# Autodesk Inventor assembly: Krasser Roboter weniger Gewindestangen
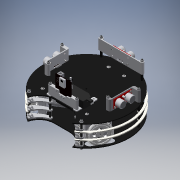
[picture p0: Inventor's stored thumbnail of the model, 180x180]
Saved by Autodesk Inventor 2018 (Build 220112000, 112)
## iProperties
Created: 2019-03-04
Part Number: Krasser Roboter weniger Gewindestangen
Material: Generisch
Document SubType Name: Assembly
Designer: RedBots
Mass: 1105.68 g
Surface Area: 3152.09 cm^2
Volume: 618.707 cm^3
Density: 1.78708 g/cm^3
Author: RedBots
## Documents named in this file (37)
- C:\Users\RedBots\Desktop\FinalRobot\Krasser Roboter weniger Gewindestangen.iam
- C:\Users\RedBots\Desktop\FinalRobot\Bodenplatine.ipt
- C:\Users\RedBots\Desktop\FinalRobot\alu_ring_pesus.ipt
- C:\Users\RedBots\Desktop\FinalRobot\Fake Rad.ipt
- C:\Users\RedBots\Desktop\FinalRobot\Hauptplatine.ipt
- C:\Users\RedBots\Desktop\FinalRobot\Akku.ipt
- C:\Users\RedBots\Desktop\FinalRobot\Akkuhalterung.ipt
- C:\Users\RedBots\Desktop\FinalRobot\Schraube M3x8 SK.ipt
- C:\Users\RedBots\Desktop\FinalRobot\Motor\Motormaxon_PN_B7453F27107C.iam
- C:\Users\RedBots\Desktop\FinalRobot\LED 3mm.ipt
- C:\Users\RedBots\Desktop\FinalRobot\Halterung Lichtschranke rechts.ipt
- C:\Users\RedBots\Desktop\FinalRobot\Ball.ipt
- C:\Users\RedBots\Desktop\FinalRobot\Halterung Lichtschranke links.ipt
- C:\Users\RedBots\Desktop\FinalRobot\SRF08.ipt
- C:\Users\RedBots\Desktop\FinalRobot\Pinhead 5.ipt
- C:\Users\RedBots\Desktop\FinalRobot\Schraube M3x8 LK.ipt
- C:\Users\RedBots\Desktop\FinalRobot\US Halterung rechts.ipt
- C:\Users\RedBots\Desktop\FinalRobot\US Halterung links.ipt
- C:\Users\RedBots\Desktop\FinalRobot\Pixy 2.iam
- C:\Users\RedBots\Desktop\FinalRobot\Pixy 2 Halterung.ipt
- C:\Users\RedBots\Desktop\FinalRobot\Abstandshalter US Sensor.ipt
- C:\Users\RedBots\Desktop\FinalRobot\Scheibe M3 Polyamid.ipt
- C:\Users\RedBots\Desktop\FinalRobot\Sicherungsmutter M3.ipt
- C:\Users\RedBots\Desktop\FinalRobot\Schraube M3x16 LK.ipt
- C:\Users\RedBots\Desktop\FinalRobot\US Halterung hinten leicht.ipt
- C:\Users\RedBots\Desktop\FinalRobot\Gewindestange M3x103mm.ipt
- C:\Users\RedBots\Desktop\FinalRobot\Abstandshalter 15mm leicht.ipt
- C:\Users\RedBots\Desktop\FinalRobot\Abstandshalter 12mm leicht.ipt
- C:\Users\RedBots\Desktop\FinalRobot\Abstandshalter 3mm.ipt
- C:\Users\RedBots\Desktop\FinalRobot\Gewindestange M3x91mm.ipt
- C:\Users\RedBots\Desktop\FinalRobot\Gewindestange M3x63mm.ipt
- C:\Users\RedBots\Desktop\FinalRobot\Abstandshalter 14mm leicht.ipt
- C:\Users\RedBots\Desktop\FinalRobot\Gewindestange M3x85mm.ipt
- C:\Users\RedBots\Desktop\FinalRobot\Schraube M3x12 LK.ipt
- C:\Users\RedBots\Desktop\FinalRobot\Motorhalterung leicht H.ipt
- C:\Users\RedBots\Desktop\FinalRobot\Motorhalterung leicht VL.ipt
- C:\Users\RedBots\Desktop\FinalRobot\Motorhalterung leicht VR.ipt
## Components (151 placed, 37 different names)
1. Ball:1 — Passend:142, Passend:143
2. Abstandshalter 3mm:1 — Passend:322, Passend:328
3. Abstandshalter 3mm:2 — Passend:330, Passend:331, Passend:332
4. Abstandshalter 3mm:3 — Passend:337, Passend:339
5. Abstandshalter 3mm:4 — Passend:338, Passend:340, Passend:341
6. Gewindestange M3x91mm:1 — Passend:323, Passend:324, Fluchtend:31, Passend:325, Passend:326, Passend:329, Passend:330, Passend:333
7. Sicherungsmutter M3:15 — Passend:326, Passend:327
8. Sicherungsmutter M3:16 — Passend:333, Passend:336
9. Sicherungsmutter M3:17 — Passend:334, Passend:335
10. Sicherungsmutter M3:18 — Passend:342, Passend:344
11. Sicherungsmutter M3:19 — Passend:343, Passend:345
12. Abstandshalter 15mm leicht:13 — Passend:347, Passend:349
13. Abstandshalter 15mm leicht:14 — Passend:346, Passend:348, Passend:350
14. Sicherungsmutter M3:20 — Passend:351, Passend:353
15. Sicherungsmutter M3:21 — Passend:352, Passend:354
16. Schraube M3x16 LK:4 — Passend:355, Passend:356, Passend:357, Passend:358
17. Schraube M3x16 LK:5 — Passend:359, Passend:360, Passend:361, Passend:362
18. Schraube M3x16 LK:6 — Passend:363, Passend:364, Passend:365
19. Schraube M3x16 LK:7 — Passend:366, Passend:367, Passend:368
20. Sicherungsmutter M3:22 — Passend:370, Passend:372
21. Sicherungsmutter M3:23 — Passend:369, Passend:371
22. Abstandshalter 12mm leicht:7 — Passend:373, Passend:375
23. Abstandshalter 12mm leicht:8 — Passend:374, Passend:376, Passend:377
24. Abstandshalter 14mm leicht:1 — Passend:380, Passend:382
25. Abstandshalter 14mm leicht:2 — Passend:379, Passend:385, Passend:387
26. Abstandshalter 14mm leicht:3 — Passend:378, Passend:384, Passend:386
27. Abstandshalter 14mm leicht:4 — Passend:381, Passend:383
28. Sicherungsmutter M3:24 — Passend:389, Passend:391
29. Sicherungsmutter M3:25 — Passend:390, Passend:392
30. Schraube M3x16 LK:8 — Passend:399, Passend:400
31. Schraube M3x16 LK:9 — Passend:393, Passend:394, Passend:397
32. Scheibe M3 Polyamid:27 — Passend:395, Passend:396, Passend:397
33. Sicherungsmutter M3:26 — Passend:405, Passend:408
34. Sicherungsmutter M3:27 — Passend:404, Passend:407
35. Sicherungsmutter M3:28 — Passend:406, Passend:409
36. Bodenplatine:1 — Passend:17, Fluchtend:2, Passend:18, Passend:21, Passend:24, Passend:25, Passend:26, Passend:27, Passend:28, Passend:29, Passend:30, Passend:31, Passend:32, Fluchtend:7, Fluchtend:8, Fluchtend:9, Fluchtend:10, Fluchtend:11, Fluchtend:12, Fluchtend:13, Fluchtend:14, Passend:100, Passend:102, Passend:105, Passend:106, Passend:143, Passend:157, Passend:158, Passend:262, Passend:263, Passend:264, Passend:265, Passend:266, Passend:267, Passend:268, Passend:269, Passend:270, Passend:271, Passend:272, Passend:273, Passend:274, Passend:275, Passend:324, Fluchtend:31, Passend:367, Passend:398
37. Hauptplatine:1 — Passend:48, Passend:49, Passend:50, Passend:53, Passend:54, Passend:61, Passend:63, Passend:238, Passend:241, Passend:243, Passend:245, Passend:247, Passend:331, Passend:339, Passend:340, Passend:348, Passend:349, Passend:355, Passend:361, Passend:375, Passend:376, Passend:394, Passend:395, Passend:396
38. Gewindestange M3x85mm:2 — Passend:28, Fluchtend:8, Passend:62, Passend:128, Passend:137, Passend:140, Passend:209, Passend:250, Passend:293, Passend:374, Passend:380, Passend:381, Passend:390
39. Gewindestange M3x85mm:1 — Passend:26, Fluchtend:9, Passend:60, Passend:130, Passend:134, Passend:138, Passend:208, Passend:261, Passend:276, Passend:373, Passend:378, Passend:379, Passend:389
40. Gewindestange M3x91mm:3 — Passend:13, Passend:17, Fluchtend:2, Passend:179, Passend:258, Passend:292, Passend:338, Passend:343
41. Gewindestange M3x63mm:1 — Passend:25, Fluchtend:10, Passend:33, Passend:36, Passend:49, Passend:86, Passend:87, Passend:112, Passend:131, Passend:135, Passend:139, Passend:234, Passend:260, Passend:298, Passend:370
42. Gewindestange M3x63mm:2 — Passend:29, Fluchtend:7, Passend:34, Passend:37, Passend:50, Passend:92, Passend:93, Passend:113, Passend:129, Passend:136, Passend:141, Passend:227, Passend:248, Passend:300, Passend:369
43. Gewindestange M3x91mm:2 — Passend:30, Fluchtend:14, Passend:94, Passend:95, Passend:114, Passend:204, Passend:252, Passend:280, Passend:322, Passend:334
44. Gewindestange M3x103mm:1 — Passend:32, Fluchtend:12, Passend:90, Passend:91, Passend:116, Passend:256, Passend:288, Passend:317, Passend:347, Passend:352
45. Gewindestange M3x103mm:2 — Passend:31, Fluchtend:13, Passend:96, Passend:97, Passend:117, Passend:253, Passend:285, Passend:316, Passend:346, Passend:351
46. Gewindestange M3x91mm:4 — Passend:27, Fluchtend:11, Passend:88, Passend:89, Passend:115, Passend:180, Passend:257, Passend:289, Passend:337, Passend:342
47. Ring unten — Passend:33, Passend:34, Passend:101, Passend:103, Passend:104, Passend:107, Passend:110, Passend:156, Passend:159
48. Ring oben — Passend:36, Passend:37, Passend:111, Passend:118, Passend:119, Passend:120, Passend:121, Passend:132, Passend:133
49. Fake Rad:1 — Tangential:2, Passend:75, Fluchtend:23
50. Fake Rad:2 — Tangential:1, Passend:70, Fluchtend:22
51. Fake Rad:3 — Passend:76, Fluchtend:24
52. Akku:1 — Passend:59, Passend:64, Fluchtend:18
53. Akkuhalterung:1 — Passend:54, Passend:62, Passend:63
54. Akkuhalterung:2 — Passend:53, Passend:59, Passend:60, Passend:61, Passend:64, Fluchtend:18, Passend:388
55. Motormaxon_PN_B7453F27107C:3 [sub-assembly] — Passend:68, Passend:69, Passend:70, Fluchtend:22, Passend:85
56. Motormaxon_PN_B7453F27107C:1 [sub-assembly] — Passend:71, Passend:72, Passend:75, Fluchtend:23, Passend:84
57. Motormaxon_PN_B7453F27107C:2 [sub-assembly] — Passend:73, Passend:74, Passend:76, Fluchtend:24, Passend:80, Passend:81, Passend:82, Passend:83
58. Abstandshalter 12mm leicht:1 — Passend:86, Passend:98
59. Abstandshalter 12mm leicht:2 — Passend:87, Passend:99
60. Abstandshalter 12mm leicht:3 — Passend:93, Passend:109
61. Abstandshalter 12mm leicht:4 — Passend:92, Passend:108, Passend:110
62. Abstandshalter 12mm leicht:5 — Passend:112, Passend:122
63. Abstandshalter 12mm leicht:6 — Passend:113, Passend:123
64. Abstandshalter 15mm leicht:1 — Passend:97, Passend:104
65. Abstandshalter 15mm leicht:2 — Passend:95, Passend:107, Passend:111
66. Abstandshalter 15mm leicht:3 — Passend:96, Passend:105
67. Abstandshalter 15mm leicht:4 — Passend:94, Passend:106
68. Abstandshalter 15mm leicht:5 — Passend:88, Passend:101
69. Abstandshalter 15mm leicht:6 — Passend:89, Passend:100
70. Abstandshalter 15mm leicht:7 — Passend:90, Passend:102
71. Abstandshalter 15mm leicht:8 — Passend:91, Passend:103
72. Abstandshalter 15mm leicht:9 — Passend:115, Passend:121
73. Abstandshalter 15mm leicht:10 — Passend:114, Passend:119
74. Abstandshalter 15mm leicht:11 — Passend:116, Passend:120
75. Abstandshalter 15mm leicht:12 — Passend:117, Passend:118
76. Halterung Lichtschranke links:1 — Passend:130, Passend:131, Passend:132, Passend:144, Passend:145, Passend:122, Passend:384
77. Halterung Lichtschranke links:2 — Passend:134, Passend:135, Passend:146, Passend:154, Passend:156, Passend:99, Passend:385, Passend:386
78. Halterung Lichtschranke rechts:2 — Passend:136, Passend:137, Passend:149, Passend:152, Passend:159, Passend:109, Passend:383
79. Halterung Lichtschranke links:3 — Passend:138, Passend:139, Passend:147, Passend:155, Passend:157, Passend:98, Passend:387
80. Halterung Lichtschranke rechts:3 — Passend:140, Passend:141, Passend:150, Passend:153, Passend:158, Passend:108
81. Halterung Lichtschranke rechts:1 — Passend:128, Passend:129, Passend:133, Passend:148, Passend:151, Passend:123, Passend:377, Passend:382
82. LED 3mm:1 — Passend:144, Passend:145
83. LED 3mm:2 — Passend:150, Passend:153
84. LED 3mm:3 — Passend:149, Passend:152
85. LED 3mm:4 — Passend:147, Passend:155
86. LED 3mm:5 — Passend:146, Passend:154
87. LED 3mm:6 — Passend:148, Passend:151
88. Schraube M3x12 LK:3 — Passend:402, Passend:406
89. Schraube M3x12 LK:2 — Passend:403, Passend:405
90. Schraube M3x12 LK:1 — Passend:401, Passend:404
91. Pixy 2 Halterung:1 — Passend:208, Passend:209, Passend:212, Passend:213, Passend:214, Passend:215, Passend:402, Passend:403, Passend:388, Passend:391, Passend:392, Passend:401, Passend:407, Passend:408, Passend:409
92. Pixy 2:2 [sub-assembly] — Passend:212, Passend:213, Passend:214, Passend:215
93. Scheibe M3 Polyamid:3 — Passend:227, Passend:243, Passend:371
94. Scheibe M3 Polyamid:4 — Passend:234, Passend:238, Passend:372
95. Scheibe M3 Polyamid:7 — Passend:247, Passend:360, Passend:362
96. Scheibe M3 Polyamid:8 — Passend:245, Passend:357, Passend:358
97. Scheibe M3 Polyamid:10 — Passend:241, Passend:315
98. Scheibe M3 Polyamid:13 — Passend:265, Passend:325, Passend:327
99. Scheibe M3 Polyamid:14 — Passend:256, Passend:270, Passend:291
100. Scheibe M3 Polyamid:15 — Passend:248, Passend:262, Passend:303
101. Scheibe M3 Polyamid:16 — Passend:263, Passend:313
102. Scheibe M3 Polyamid:17 — Passend:260, Passend:275, Passend:301
103. Scheibe M3 Polyamid:18 — Passend:261, Passend:273, Passend:277
104. Scheibe M3 Polyamid:19 — Passend:258, Passend:272, Passend:295
105. Scheibe M3 Polyamid:20 — Passend:268, Passend:364, Passend:365
106. Scheibe M3 Polyamid:21 — Passend:269, Passend:366, Passend:368
107. Scheibe M3 Polyamid:22 — Passend:253, Passend:267, Passend:287
108. Scheibe M3 Polyamid:23 — Passend:274, Passend:398, Passend:399, Passend:400
109. Scheibe M3 Polyamid:24 — Passend:257, Passend:271, Passend:290
110. Scheibe M3 Polyamid:25 — Passend:252, Passend:266, Passend:282
111. Scheibe M3 Polyamid:26 — Passend:250, Passend:264, Passend:294
112. Sicherungsmutter M3:1 — Passend:288, Passend:291
113. Sicherungsmutter M3:2 — Passend:289, Passend:290
114. Sicherungsmutter M3:4 — Passend:285, Passend:287
115. Sicherungsmutter M3:6 — Passend:276, Passend:277
116. Sicherungsmutter M3:7 — Passend:280, Passend:282
117. Sicherungsmutter M3:10 — Passend:293, Passend:294
118. Sicherungsmutter M3:11 — Passend:292, Passend:295
119. Sicherungsmutter M3:12 — Passend:298, Passend:301
120. Sicherungsmutter M3:14 — Passend:300, Passend:303
121. Schraube M3x8 SK:1 — Fluchtend:19, Passend:67
122. Schraube M3x8 SK:2 — Fluchtend:20, Passend:66
123. Schraube M3x8 SK:3 — Fluchtend:21, Passend:65
124. Motorhalterung leicht VR:1 — Passend:13, Passend:18, Fluchtend:19, Fluchtend:20, Fluchtend:21, Passend:65, Passend:66, Passend:67, Passend:71, Passend:72, Passend:84, Passend:393
125. Motorhalterung leicht H:1 — Passend:24, Passend:68, Passend:69, Passend:77, Passend:78, Passend:79, Fluchtend:25, Fluchtend:26, Fluchtend:27, Passend:85, Passend:356, Passend:359, Passend:363
126. Schraube M3x8 SK:4 — Passend:77, Fluchtend:26
127. Schraube M3x8 SK:5 — Passend:78, Fluchtend:27
128. Schraube M3x8 SK:6 — Passend:79, Fluchtend:25
129. Schraube M3x16 LK:1 — Passend:313
130. Schraube M3x16 LK:3 — Passend:314, Passend:315
131. Motorhalterung leicht VL:1 — Passend:21, Passend:48, Passend:73, Passend:74, Passend:83, Fluchtend:28, Fluchtend:29, Fluchtend:30, Passend:314, Passend:323
132. Schraube M3x8 SK:7 — Passend:81, Fluchtend:28
133. Schraube M3x8 SK:8 — Passend:82, Fluchtend:30
134. Schraube M3x8 SK:9 — Passend:80, Fluchtend:29
135. Pinhead 5:1 — Passend:164, Passend:165, Passend:166
136. SRF08:3 — Passend:164, Passend:165, Passend:166, Passend:172, Passend:173, Passend:174, Passend:175, Passend:224, Passend:225
137. US Halterung hinten leicht:1 — Passend:316, Passend:317, Passend:319, Passend:320, Passend:321, Passend:350, Passend:353, Passend:354
138. Schraube M3x8 LK:1 — Passend:173, Passend:174, Passend:223, Passend:320
139. Schraube M3x8 LK:2 — Passend:172, Passend:175, Passend:222, Passend:319
140. Abstandshalter US Sensor:1 — Passend:222, Passend:224, Passend:321
141. Abstandshalter US Sensor:2 — Passend:223, Passend:225
142. SRF08:2 — Passend:182, Passend:183, Passend:184, Passend:185, Passend:186, Passend:187, Passend:188, Passend:189
143. US Halterung rechts:1 — Passend:179, Passend:180, Passend:182, Passend:190, Passend:191, Passend:341, Passend:344, Passend:345
144. Pinhead 5:2 — Passend:183, Passend:184, Passend:185
145. Schraube M3x8 LK:3 — Passend:186, Passend:188, Passend:191
146. Schraube M3x8 LK:4 — Passend:187, Passend:189, Passend:190
147. SRF08:1 — Passend:195, Passend:196, Passend:197, Passend:198, Passend:199, Passend:200, Passend:201, Passend:205
148. Pinhead 5:3 — Passend:195, Passend:196, Passend:197
149. Schraube M3x8 LK:5 — Passend:199, Passend:201, Passend:207
150. Schraube M3x8 LK:6 — Passend:198, Passend:200, Passend:206
151. US Halterung links:1 — Passend:204, Passend:205, Passend:206, Passend:207, Passend:328, Passend:329, Passend:332, Passend:335, Passend:336
## Relationships (334: Mate 309, Flush 23, Tangent 2)
- Passend:13 [Mate]: Gewindestange M3x91mm:3 ↔ Motorhalterung leicht VR:1
- Passend:17 [Mate]: Bodenplatine:1 ↔ Gewindestange M3x91mm:3
- Fluchtend:2 [Flush] (-5 mm): Bodenplatine:1 ↔ Gewindestange M3x91mm:3
- Passend:18 [Mate]: Bodenplatine:1 ↔ Motorhalterung leicht VR:1
- Passend:21 [Mate]: Bodenplatine:1 ↔ Motorhalterung leicht VL:1
- Passend:24 [Mate]: Bodenplatine:1 ↔ Motorhalterung leicht H:1
- Passend:25 [Mate]: Bodenplatine:1 ↔ Gewindestange M3x63mm:1
- Passend:26 [Mate]: Bodenplatine:1 ↔ Gewindestange M3x85mm:1
- Passend:27 [Mate]: Bodenplatine:1 ↔ Gewindestange M3x91mm:4
- Passend:28 [Mate]: Bodenplatine:1 ↔ Gewindestange M3x85mm:2
- Passend:29 [Mate]: Bodenplatine:1 ↔ Gewindestange M3x63mm:2
- Passend:30 [Mate]: Bodenplatine:1 ↔ Gewindestange M3x91mm:2
- Passend:31 [Mate]: Bodenplatine:1 ↔ Gewindestange M3x103mm:2
- Passend:32 [Mate]: Bodenplatine:1 ↔ Gewindestange M3x103mm:1
- Fluchtend:7 [Flush] (-5 mm): Bodenplatine:1 ↔ Gewindestange M3x63mm:2
- Fluchtend:8 [Flush] (5 mm): Bodenplatine:1 ↔ Gewindestange M3x85mm:2
- Fluchtend:9 [Flush] (5 mm): Bodenplatine:1 ↔ Gewindestange M3x85mm:1
- Fluchtend:10 [Flush] (5 mm): Bodenplatine:1 ↔ Gewindestange M3x63mm:1
- Fluchtend:11 [Flush] (-5 mm): Bodenplatine:1 ↔ Gewindestange M3x91mm:4
- Fluchtend:12 [Flush] (-5 mm): Bodenplatine:1 ↔ Gewindestange M3x103mm:1
- Fluchtend:13 [Flush] (-5 mm): Bodenplatine:1 ↔ Gewindestange M3x103mm:2
- Fluchtend:14 [Flush] (-5 mm): Bodenplatine:1 ↔ Gewindestange M3x91mm:2
- Passend:33 [Mate]: Gewindestange M3x63mm:1 ↔ Ring unten
- Passend:34 [Mate]: Gewindestange M3x63mm:2 ↔ Ring unten
- Passend:36 [Mate]: Gewindestange M3x63mm:1 ↔ Ring oben
- Passend:37 [Mate]: Gewindestange M3x63mm:2 ↔ Ring oben
- Passend:48 [Mate]: Hauptplatine:1 ↔ Motorhalterung leicht VL:1
- Passend:49 [Mate]: Hauptplatine:1 ↔ Gewindestange M3x63mm:1
- Passend:50 [Mate]: Hauptplatine:1 ↔ Gewindestange M3x63mm:2
- Passend:53 [Mate]: Hauptplatine:1 ↔ Akkuhalterung:2
- Passend:54 [Mate]: Hauptplatine:1 ↔ Akkuhalterung:1
- Passend:59 [Mate]: Akku:1 ↔ Akkuhalterung:2
- Passend:60 [Mate]: Gewindestange M3x85mm:1 ↔ Akkuhalterung:2
- Passend:61 [Mate]: Hauptplatine:1 ↔ Akkuhalterung:2
- Passend:62 [Mate]: Gewindestange M3x85mm:2 ↔ Akkuhalterung:1
- Passend:63 [Mate]: Hauptplatine:1 ↔ Akkuhalterung:1
- Tangential:1: Fake Rad:2
- Tangential:2: Fake Rad:1
- Passend:64 [Mate] (1.5 mm): Akku:1 ↔ Akkuhalterung:2
- Fluchtend:18 [Flush]: Akku:1 ↔ Akkuhalterung:2
- Fluchtend:19 [Flush]: Schraube M3x8 SK:1 ↔ Motorhalterung leicht VR:1
- Fluchtend:20 [Flush]: Schraube M3x8 SK:2 ↔ Motorhalterung leicht VR:1
- Fluchtend:21 [Flush]: Schraube M3x8 SK:3 ↔ Motorhalterung leicht VR:1
- Passend:65 [Mate]: Schraube M3x8 SK:3 ↔ Motorhalterung leicht VR:1
- Passend:66 [Mate]: Schraube M3x8 SK:2 ↔ Motorhalterung leicht VR:1
- Passend:67 [Mate]: Schraube M3x8 SK:1 ↔ Motorhalterung leicht VR:1
- Passend:68 [Mate]: Motormaxon_PN_B7453F27107C:3 ↔ Motorhalterung leicht H:1
- Passend:69 [Mate]: Motormaxon_PN_B7453F27107C:3 ↔ Motorhalterung leicht H:1
- Passend:70 [Mate]: Fake Rad:2 ↔ Motormaxon_PN_B7453F27107C:3
- Fluchtend:22 [Flush] (-0.5 mm): Fake Rad:2 ↔ Motormaxon_PN_B7453F27107C:3
- Passend:71 [Mate]: Motormaxon_PN_B7453F27107C:1 ↔ Motorhalterung leicht VR:1
- Passend:72 [Mate]: Motormaxon_PN_B7453F27107C:1 ↔ Motorhalterung leicht VR:1
- Passend:73 [Mate]: Motormaxon_PN_B7453F27107C:2 ↔ Motorhalterung leicht VL:1
- Passend:74 [Mate]: Motormaxon_PN_B7453F27107C:2 ↔ Motorhalterung leicht VL:1
- Passend:75 [Mate]: Fake Rad:1 ↔ Motormaxon_PN_B7453F27107C:1
- Fluchtend:23 [Flush] (0.5 mm): Fake Rad:1 ↔ Motormaxon_PN_B7453F27107C:1
- Passend:76 [Mate]: Fake Rad:3 ↔ Motormaxon_PN_B7453F27107C:2
- Fluchtend:24 [Flush] (-0.5 mm): Fake Rad:3 ↔ Motormaxon_PN_B7453F27107C:2
- Passend:77 [Mate]: Motorhalterung leicht H:1 ↔ Schraube M3x8 SK:4
- Passend:78 [Mate]: Motorhalterung leicht H:1 ↔ Schraube M3x8 SK:5
- Passend:79 [Mate]: Motorhalterung leicht H:1 ↔ Schraube M3x8 SK:6
- Fluchtend:25 [Flush]: Motorhalterung leicht H:1 ↔ Schraube M3x8 SK:6
- Fluchtend:26 [Flush]: Motorhalterung leicht H:1 ↔ Schraube M3x8 SK:4
- Fluchtend:27 [Flush]: Motorhalterung leicht H:1 ↔ Schraube M3x8 SK:5
- Passend:80 [Mate]: Motormaxon_PN_B7453F27107C:2 ↔ Schraube M3x8 SK:9
- Passend:81 [Mate]: Motormaxon_PN_B7453F27107C:2 ↔ Schraube M3x8 SK:7
- Passend:82 [Mate]: Motormaxon_PN_B7453F27107C:2 ↔ Schraube M3x8 SK:8
- Passend:83 [Mate]: Motormaxon_PN_B7453F27107C:2 ↔ Motorhalterung leicht VL:1
- Fluchtend:28 [Flush]: Motorhalterung leicht VL:1 ↔ Schraube M3x8 SK:7
- Fluchtend:29 [Flush]: Motorhalterung leicht VL:1 ↔ Schraube M3x8 SK:9
- Fluchtend:30 [Flush]: Motorhalterung leicht VL:1 ↔ Schraube M3x8 SK:8
- Passend:84 [Mate]: Motormaxon_PN_B7453F27107C:1 ↔ Motorhalterung leicht VR:1
- Passend:85 [Mate]: Motormaxon_PN_B7453F27107C:3 ↔ Motorhalterung leicht H:1
- Passend:86 [Mate]: Gewindestange M3x63mm:1 ↔ Abstandshalter 12mm leicht:1
- Passend:87 [Mate]: Gewindestange M3x63mm:1 ↔ Abstandshalter 12mm leicht:2
- Passend:88 [Mate]: Gewindestange M3x91mm:4 ↔ Abstandshalter 15mm leicht:5
- Passend:89 [Mate]: Gewindestange M3x91mm:4 ↔ Abstandshalter 15mm leicht:6
- Passend:90 [Mate]: Gewindestange M3x103mm:1 ↔ Abstandshalter 15mm leicht:7
- Passend:91 [Mate]: Gewindestange M3x103mm:1 ↔ Abstandshalter 15mm leicht:8
- Passend:92 [Mate]: Gewindestange M3x63mm:2 ↔ Abstandshalter 12mm leicht:4
- Passend:93 [Mate]: Gewindestange M3x63mm:2 ↔ Abstandshalter 12mm leicht:3
- Passend:94 [Mate]: Gewindestange M3x91mm:2 ↔ Abstandshalter 15mm leicht:4
- Passend:95 [Mate]: Gewindestange M3x91mm:2 ↔ Abstandshalter 15mm leicht:2
- Passend:96 [Mate]: Gewindestange M3x103mm:2 ↔ Abstandshalter 15mm leicht:3
- Passend:97 [Mate]: Gewindestange M3x103mm:2 ↔ Abstandshalter 15mm leicht:1
- Passend:98 [Mate]: Abstandshalter 12mm leicht:1 ↔ Halterung Lichtschranke links:3
- Passend:99 [Mate]: Abstandshalter 12mm leicht:2 ↔ Halterung Lichtschranke links:2
- Passend:100 [Mate]: Bodenplatine:1 ↔ Abstandshalter 15mm leicht:6
- Passend:101 [Mate]: Ring unten ↔ Abstandshalter 15mm leicht:5
- Passend:102 [Mate]: Bodenplatine:1 ↔ Abstandshalter 15mm leicht:7
- Passend:103 [Mate]: Ring unten ↔ Abstandshalter 15mm leicht:8
- Passend:104 [Mate]: Ring unten ↔ Abstandshalter 15mm leicht:1
- Passend:105 [Mate]: Bodenplatine:1 ↔ Abstandshalter 15mm leicht:3
- Passend:106 [Mate]: Bodenplatine:1 ↔ Abstandshalter 15mm leicht:4
- Passend:107 [Mate]: Ring unten ↔ Abstandshalter 15mm leicht:2
- Passend:108 [Mate]: Abstandshalter 12mm leicht:4 ↔ Halterung Lichtschranke rechts:3
- Passend:109 [Mate]: Abstandshalter 12mm leicht:3 ↔ Halterung Lichtschranke rechts:2
- Passend:110 [Mate]: Ring unten ↔ Abstandshalter 12mm leicht:4
- Passend:111 [Mate]: Ring oben ↔ Abstandshalter 15mm leicht:2
- Passend:112 [Mate]: Gewindestange M3x63mm:1 ↔ Abstandshalter 12mm leicht:5
- Passend:113 [Mate]: Gewindestange M3x63mm:2 ↔ Abstandshalter 12mm leicht:6
- Passend:114 [Mate]: Gewindestange M3x91mm:2 ↔ Abstandshalter 15mm leicht:10
- Passend:115 [Mate]: Gewindestange M3x91mm:4 ↔ Abstandshalter 15mm leicht:9
- Passend:116 [Mate]: Gewindestange M3x103mm:1 ↔ Abstandshalter 15mm leicht:11
- Passend:117 [Mate]: Gewindestange M3x103mm:2 ↔ Abstandshalter 15mm leicht:12
- Passend:118 [Mate]: Ring oben ↔ Abstandshalter 15mm leicht:12
- Passend:119 [Mate]: Ring oben ↔ Abstandshalter 15mm leicht:10
- Passend:120 [Mate]: Ring oben ↔ Abstandshalter 15mm leicht:11
- Passend:121 [Mate]: Ring oben ↔ Abstandshalter 15mm leicht:9
- Passend:122 [Mate]: Abstandshalter 12mm leicht:5 ↔ Halterung Lichtschranke links:1
- Passend:123 [Mate]: Abstandshalter 12mm leicht:6 ↔ Halterung Lichtschranke rechts:1
- Passend:128 [Mate]: Gewindestange M3x85mm:2 ↔ Halterung Lichtschranke rechts:1
- Passend:129 [Mate]: Gewindestange M3x63mm:2 ↔ Halterung Lichtschranke rechts:1
- Passend:130 [Mate]: Gewindestange M3x85mm:1 ↔ Halterung Lichtschranke links:1
- Passend:131 [Mate]: Gewindestange M3x63mm:1 ↔ Halterung Lichtschranke links:1
- Passend:132 [Mate]: Ring oben ↔ Halterung Lichtschranke links:1
- Passend:133 [Mate]: Ring oben ↔ Halterung Lichtschranke rechts:1
- Passend:134 [Mate]: Gewindestange M3x85mm:1 ↔ Halterung Lichtschranke links:2
- Passend:135 [Mate]: Gewindestange M3x63mm:1 ↔ Halterung Lichtschranke links:2
- Passend:136 [Mate]: Gewindestange M3x63mm:2 ↔ Halterung Lichtschranke rechts:2
- Passend:137 [Mate]: Gewindestange M3x85mm:2 ↔ Halterung Lichtschranke rechts:2
- Passend:138 [Mate]: Gewindestange M3x85mm:1 ↔ Halterung Lichtschranke links:3
- Passend:139 [Mate]: Gewindestange M3x63mm:1 ↔ Halterung Lichtschranke links:3
- Passend:140 [Mate]: Gewindestange M3x85mm:2 ↔ Halterung Lichtschranke rechts:3
- Passend:141 [Mate]: Gewindestange M3x63mm:2 ↔ Halterung Lichtschranke rechts:3
- Passend:142 [Mate] (37 mm): Ball:1
- Passend:143 [Mate] (37 mm): Ball:1 ↔ Bodenplatine:1
- Passend:144 [Mate]: Halterung Lichtschranke links:1 ↔ LED 3mm:1
- Passend:145 [Mate]: Halterung Lichtschranke links:1 ↔ LED 3mm:1
- Passend:146 [Mate]: Halterung Lichtschranke links:2 ↔ LED 3mm:5
- Passend:147 [Mate]: Halterung Lichtschranke links:3 ↔ LED 3mm:4
- Passend:148 [Mate]: Halterung Lichtschranke rechts:1 ↔ LED 3mm:6
- Passend:149 [Mate]: Halterung Lichtschranke rechts:2 ↔ LED 3mm:3
- Passend:150 [Mate]: Halterung Lichtschranke rechts:3 ↔ LED 3mm:2
- Passend:151 [Mate]: Halterung Lichtschranke rechts:1 ↔ LED 3mm:6
- Passend:152 [Mate]: Halterung Lichtschranke rechts:2 ↔ LED 3mm:3
- Passend:153 [Mate]: Halterung Lichtschranke rechts:3 ↔ LED 3mm:2
- Passend:154 [Mate]: Halterung Lichtschranke links:2 ↔ LED 3mm:5
- Passend:155 [Mate]: Halterung Lichtschranke links:3 ↔ LED 3mm:4
- Passend:156 [Mate]: Ring unten ↔ Halterung Lichtschranke links:2
- Passend:157 [Mate]: Bodenplatine:1 ↔ Halterung Lichtschranke links:3
- Passend:158 [Mate]: Bodenplatine:1 ↔ Halterung Lichtschranke rechts:3
- Passend:159 [Mate]: Ring unten ↔ Halterung Lichtschranke rechts:2
- Passend:164 [Mate]: Pinhead 5:1 ↔ SRF08:3
- Passend:165 [Mate]: Pinhead 5:1 ↔ SRF08:3
- Passend:166 [Mate]: Pinhead 5:1 ↔ SRF08:3
- Passend:172 [Mate]: SRF08:3 ↔ Schraube M3x8 LK:2
- Passend:173 [Mate]: SRF08:3 ↔ Schraube M3x8 LK:1
- Passend:174 [Mate]: SRF08:3 ↔ Schraube M3x8 LK:1
- Passend:175 [Mate]: SRF08:3 ↔ Schraube M3x8 LK:2
- Passend:179 [Mate]: Gewindestange M3x91mm:3 ↔ US Halterung rechts:1
- Passend:180 [Mate]: Gewindestange M3x91mm:4 ↔ US Halterung rechts:1
- Passend:182 [Mate]: SRF08:2 ↔ US Halterung rechts:1
- Passend:183 [Mate]: SRF08:2 ↔ Pinhead 5:2
- Passend:184 [Mate]: SRF08:2 ↔ Pinhead 5:2
- Passend:185 [Mate]: SRF08:2 ↔ Pinhead 5:2
- Passend:186 [Mate]: SRF08:2 ↔ Schraube M3x8 LK:3
- Passend:187 [Mate]: SRF08:2 ↔ Schraube M3x8 LK:4
- Passend:188 [Mate]: SRF08:2 ↔ Schraube M3x8 LK:3
- Passend:189 [Mate]: SRF08:2 ↔ Schraube M3x8 LK:4
- Passend:190 [Mate]: US Halterung rechts:1 ↔ Schraube M3x8 LK:4
- Passend:191 [Mate]: US Halterung rechts:1 ↔ Schraube M3x8 LK:3
- Passend:195 [Mate]: SRF08:1 ↔ Pinhead 5:3
- Passend:196 [Mate]: SRF08:1 ↔ Pinhead 5:3
- Passend:197 [Mate]: SRF08:1 ↔ Pinhead 5:3
- Passend:198 [Mate]: SRF08:1 ↔ Schraube M3x8 LK:6
- Passend:199 [Mate]: SRF08:1 ↔ Schraube M3x8 LK:5
- Passend:200 [Mate]: SRF08:1 ↔ Schraube M3x8 LK:6
- Passend:201 [Mate]: SRF08:1 ↔ Schraube M3x8 LK:5
- Passend:204 [Mate]: Gewindestange M3x91mm:2 ↔ US Halterung links:1
- Passend:205 [Mate]: SRF08:1 ↔ US Halterung links:1
- Passend:206 [Mate]: Schraube M3x8 LK:6 ↔ US Halterung links:1
- Passend:207 [Mate]: Schraube M3x8 LK:5 ↔ US Halterung links:1
- Passend:208 [Mate]: Gewindestange M3x85mm:1 ↔ Pixy 2 Halterung:1
- Passend:209 [Mate]: Gewindestange M3x85mm:2 ↔ Pixy 2 Halterung:1
- Passend:212 [Mate]: Pixy 2 Halterung:1 ↔ Pixy 2:2
- Passend:213 [Mate]: Pixy 2 Halterung:1 ↔ Pixy 2:2
- Passend:214 [Mate]: Pixy 2 Halterung:1 ↔ Pixy 2:2
- Passend:215 [Mate]: Pixy 2 Halterung:1 ↔ Pixy 2:2
- [Mate]: Schraube M3x12 LK:1 ↔ Pixy 2 Halterung:1
- [Mate]: Schraube M3x12 LK:2 ↔ Pixy 2 Halterung:1
- [Mate]: Schraube M3x12 LK:3 ↔ Pixy 2 Halterung:1
- Passend:402 [Mate]: Schraube M3x12 LK:3 ↔ Pixy 2 Halterung:1
- Passend:403 [Mate]: Schraube M3x12 LK:2 ↔ Pixy 2 Halterung:1
- Passend:222 [Mate]: Schraube M3x8 LK:2 ↔ Abstandshalter US Sensor:1
- Passend:223 [Mate]: Schraube M3x8 LK:1 ↔ Abstandshalter US Sensor:2
- Passend:224 [Mate]: SRF08:3 ↔ Abstandshalter US Sensor:1
- Passend:225 [Mate]: SRF08:3 ↔ Abstandshalter US Sensor:2
- Passend:227 [Mate]: Gewindestange M3x63mm:2 ↔ Scheibe M3 Polyamid:3
- Passend:234 [Mate]: Gewindestange M3x63mm:1 ↔ Scheibe M3 Polyamid:4
- Passend:238 [Mate]: Hauptplatine:1 ↔ Scheibe M3 Polyamid:4
- Passend:241 [Mate]: Hauptplatine:1 ↔ Scheibe M3 Polyamid:10
- Passend:243 [Mate]: Hauptplatine:1 ↔ Scheibe M3 Polyamid:3
- Passend:245 [Mate]: Hauptplatine:1 ↔ Scheibe M3 Polyamid:8
- Passend:247 [Mate]: Hauptplatine:1 ↔ Scheibe M3 Polyamid:7
- Passend:248 [Mate]: Gewindestange M3x63mm:2 ↔ Scheibe M3 Polyamid:15
- Passend:250 [Mate]: Gewindestange M3x85mm:2 ↔ Scheibe M3 Polyamid:26
- Passend:252 [Mate]: Gewindestange M3x91mm:2 ↔ Scheibe M3 Polyamid:25
- Passend:253 [Mate]: Gewindestange M3x103mm:2 ↔ Scheibe M3 Polyamid:22
- Passend:256 [Mate]: Gewindestange M3x103mm:1 ↔ Scheibe M3 Polyamid:14
- Passend:257 [Mate]: Gewindestange M3x91mm:4 ↔ Scheibe M3 Polyamid:24
- Passend:258 [Mate]: Gewindestange M3x91mm:3 ↔ Scheibe M3 Polyamid:19
- Passend:260 [Mate]: Gewindestange M3x63mm:1 ↔ Scheibe M3 Polyamid:17
- Passend:261 [Mate]: Gewindestange M3x85mm:1 ↔ Scheibe M3 Polyamid:18
- Passend:262 [Mate]: Bodenplatine:1 ↔ Scheibe M3 Polyamid:15
- Passend:263 [Mate]: Bodenplatine:1 ↔ Scheibe M3 Polyamid:16
- Passend:264 [Mate]: Bodenplatine:1 ↔ Scheibe M3 Polyamid:26
- Passend:265 [Mate]: Bodenplatine:1 ↔ Scheibe M3 Polyamid:13
- Passend:266 [Mate]: Bodenplatine:1 ↔ Scheibe M3 Polyamid:25
- Passend:267 [Mate]: Bodenplatine:1 ↔ Scheibe M3 Polyamid:22
- Passend:268 [Mate]: Bodenplatine:1 ↔ Scheibe M3 Polyamid:20
- Passend:269 [Mate]: Bodenplatine:1 ↔ Scheibe M3 Polyamid:21
- Passend:270 [Mate]: Bodenplatine:1 ↔ Scheibe M3 Polyamid:14
- Passend:271 [Mate]: Bodenplatine:1 ↔ Scheibe M3 Polyamid:24
- Passend:272 [Mate]: Bodenplatine:1 ↔ Scheibe M3 Polyamid:19
- Passend:273 [Mate]: Bodenplatine:1 ↔ Scheibe M3 Polyamid:18
- Passend:274 [Mate]: Bodenplatine:1 ↔ Scheibe M3 Polyamid:23
- Passend:275 [Mate]: Bodenplatine:1 ↔ Scheibe M3 Polyamid:17
- Passend:276 [Mate]: Gewindestange M3x85mm:1 ↔ Sicherungsmutter M3:6
- Passend:277 [Mate]: Scheibe M3 Polyamid:18 ↔ Sicherungsmutter M3:6
- Passend:280 [Mate]: Gewindestange M3x91mm:2 ↔ Sicherungsmutter M3:7
- Passend:282 [Mate]: Scheibe M3 Polyamid:25 ↔ Sicherungsmutter M3:7
- Passend:285 [Mate]: Gewindestange M3x103mm:2 ↔ Sicherungsmutter M3:4
- Passend:287 [Mate]: Scheibe M3 Polyamid:22 ↔ Sicherungsmutter M3:4
- Passend:288 [Mate]: Gewindestange M3x103mm:1 ↔ Sicherungsmutter M3:1
- Passend:289 [Mate]: Gewindestange M3x91mm:4 ↔ Sicherungsmutter M3:2
- Passend:290 [Mate]: Scheibe M3 Polyamid:24 ↔ Sicherungsmutter M3:2
- Passend:291 [Mate]: Scheibe M3 Polyamid:14 ↔ Sicherungsmutter M3:1
- Passend:292 [Mate]: Gewindestange M3x91mm:3 ↔ Sicherungsmutter M3:11
- Passend:293 [Mate]: Gewindestange M3x85mm:2 ↔ Sicherungsmutter M3:10
- Passend:294 [Mate]: Scheibe M3 Polyamid:26 ↔ Sicherungsmutter M3:10
- Passend:295 [Mate]: Scheibe M3 Polyamid:19 ↔ Sicherungsmutter M3:11
- Passend:298 [Mate]: Gewindestange M3x63mm:1 ↔ Sicherungsmutter M3:12
- Passend:300 [Mate]: Gewindestange M3x63mm:2 ↔ Sicherungsmutter M3:14
- Passend:301 [Mate]: Scheibe M3 Polyamid:17 ↔ Sicherungsmutter M3:12
- Passend:303 [Mate]: Scheibe M3 Polyamid:15 ↔ Sicherungsmutter M3:14
- [Mate]: Schraube M3x16 LK:1 ↔ Motorhalterung leicht VL:1
- [Mate]: Scheibe M3 Polyamid:16 ↔ Schraube M3x16 LK:1
- [Mate]: Bodenplatine:1 ↔ Schraube M3x16 LK:1
- Passend:313 [Mate]: Scheibe M3 Polyamid:16 ↔ Schraube M3x16 LK:1
- Passend:314 [Mate]: Schraube M3x16 LK:3 ↔ Motorhalterung leicht VL:1
- Passend:315 [Mate]: Scheibe M3 Polyamid:10 ↔ Schraube M3x16 LK:3
- Passend:316 [Mate]: Gewindestange M3x103mm:2 ↔ US Halterung hinten leicht:1
- Passend:317 [Mate]: Gewindestange M3x103mm:1 ↔ US Halterung hinten leicht:1
- Passend:319 [Mate]: US Halterung hinten leicht:1 ↔ Schraube M3x8 LK:2
- Passend:320 [Mate]: US Halterung hinten leicht:1 ↔ Schraube M3x8 LK:1
- Passend:321 [Mate]: US Halterung hinten leicht:1 ↔ Abstandshalter US Sensor:1
- Passend:322 [Mate]: Abstandshalter 3mm:1 ↔ Gewindestange M3x91mm:2
- Passend:323 [Mate]: Gewindestange M3x91mm:1 ↔ Motorhalterung leicht VL:1
- Passend:324 [Mate]: Gewindestange M3x91mm:1 ↔ Bodenplatine:1
- Fluchtend:31 [Flush] (-5 mm): Gewindestange M3x91mm:1 ↔ Bodenplatine:1
- Passend:325 [Mate]: Gewindestange M3x91mm:1 ↔ Scheibe M3 Polyamid:13
- Passend:326 [Mate]: Gewindestange M3x91mm:1 ↔ Sicherungsmutter M3:15
- Passend:327 [Mate]: Sicherungsmutter M3:15 ↔ Scheibe M3 Polyamid:13
- Passend:328 [Mate]: Abstandshalter 3mm:1 ↔ US Halterung links:1
- Passend:329 [Mate]: Gewindestange M3x91mm:1 ↔ US Halterung links:1
- Passend:330 [Mate]: Abstandshalter 3mm:2 ↔ Gewindestange M3x91mm:1
- Passend:331 [Mate]: Abstandshalter 3mm:2 ↔ Hauptplatine:1
- Passend:332 [Mate]: Abstandshalter 3mm:2 ↔ US Halterung links:1
- Passend:333 [Mate]: Gewindestange M3x91mm:1 ↔ Sicherungsmutter M3:16
- Passend:334 [Mate]: Sicherungsmutter M3:17 ↔ Gewindestange M3x91mm:2
- Passend:335 [Mate]: Sicherungsmutter M3:17 ↔ US Halterung links:1
- Passend:336 [Mate]: Sicherungsmutter M3:16 ↔ US Halterung links:1
- Passend:337 [Mate]: Abstandshalter 3mm:3 ↔ Gewindestange M3x91mm:4
- Passend:338 [Mate]: Abstandshalter 3mm:4 ↔ Gewindestange M3x91mm:3
- Passend:339 [Mate]: Abstandshalter 3mm:3 ↔ Hauptplatine:1
- Passend:340 [Mate]: Abstandshalter 3mm:4 ↔ Hauptplatine:1
- Passend:341 [Mate]: Abstandshalter 3mm:4 ↔ US Halterung rechts:1
- Passend:342 [Mate]: Sicherungsmutter M3:18 ↔ Gewindestange M3x91mm:4
- Passend:343 [Mate]: Sicherungsmutter M3:19 ↔ Gewindestange M3x91mm:3
- Passend:344 [Mate]: Sicherungsmutter M3:18 ↔ US Halterung rechts:1
- Passend:345 [Mate]: Sicherungsmutter M3:19 ↔ US Halterung rechts:1
- Passend:346 [Mate]: Abstandshalter 15mm leicht:14 ↔ Gewindestange M3x103mm:2
- Passend:347 [Mate]: Abstandshalter 15mm leicht:13 ↔ Gewindestange M3x103mm:1
- Passend:348 [Mate]: Abstandshalter 15mm leicht:14 ↔ Hauptplatine:1
- Passend:349 [Mate]: Abstandshalter 15mm leicht:13 ↔ Hauptplatine:1
- Passend:350 [Mate]: Abstandshalter 15mm leicht:14 ↔ US Halterung hinten leicht:1
- Passend:351 [Mate]: Sicherungsmutter M3:20 ↔ Gewindestange M3x103mm:2
- Passend:352 [Mate]: Sicherungsmutter M3:21 ↔ Gewindestange M3x103mm:1
- Passend:353 [Mate]: Sicherungsmutter M3:20 ↔ US Halterung hinten leicht:1
- Passend:354 [Mate]: Sicherungsmutter M3:21 ↔ US Halterung hinten leicht:1
- Passend:355 [Mate]: Schraube M3x16 LK:4 ↔ Hauptplatine:1
- Passend:356 [Mate]: Schraube M3x16 LK:4 ↔ Motorhalterung leicht H:1
- Passend:357 [Mate]: Schraube M3x16 LK:4 ↔ Scheibe M3 Polyamid:8
- Passend:358 [Mate]: Schraube M3x16 LK:4 ↔ Scheibe M3 Polyamid:8
- Passend:359 [Mate]: Schraube M3x16 LK:5 ↔ Motorhalterung leicht H:1
- Passend:360 [Mate]: Schraube M3x16 LK:5 ↔ Scheibe M3 Polyamid:7
- Passend:361 [Mate]: Schraube M3x16 LK:5 ↔ Hauptplatine:1
- Passend:362 [Mate]: Schraube M3x16 LK:5 ↔ Scheibe M3 Polyamid:7
- Passend:363 [Mate]: Schraube M3x16 LK:6 ↔ Motorhalterung leicht H:1
- Passend:364 [Mate]: Schraube M3x16 LK:6 ↔ Scheibe M3 Polyamid:20
- Passend:365 [Mate]: Schraube M3x16 LK:6 ↔ Scheibe M3 Polyamid:20
- Passend:366 [Mate]: Schraube M3x16 LK:7 ↔ Scheibe M3 Polyamid:21
- Passend:367 [Mate]: Schraube M3x16 LK:7 ↔ Bodenplatine:1
- Passend:368 [Mate]: Schraube M3x16 LK:7 ↔ Scheibe M3 Polyamid:21
- Passend:369 [Mate]: Sicherungsmutter M3:23 ↔ Gewindestange M3x63mm:2
- Passend:370 [Mate]: Sicherungsmutter M3:22 ↔ Gewindestange M3x63mm:1
- Passend:371 [Mate]: Sicherungsmutter M3:23 ↔ Scheibe M3 Polyamid:3
- Passend:372 [Mate]: Sicherungsmutter M3:22 ↔ Scheibe M3 Polyamid:4
- Passend:373 [Mate]: Abstandshalter 12mm leicht:7 ↔ Gewindestange M3x85mm:1
- Passend:374 [Mate]: Abstandshalter 12mm leicht:8 ↔ Gewindestange M3x85mm:2
- Passend:375 [Mate]: Abstandshalter 12mm leicht:7 ↔ Hauptplatine:1
- Passend:376 [Mate]: Abstandshalter 12mm leicht:8 ↔ Hauptplatine:1
- Passend:377 [Mate]: Abstandshalter 12mm leicht:8 ↔ Halterung Lichtschranke rechts:1
- Passend:378 [Mate]: Abstandshalter 14mm leicht:3 ↔ Gewindestange M3x85mm:1
- Passend:379 [Mate]: Abstandshalter 14mm leicht:2 ↔ Gewindestange M3x85mm:1
- Passend:380 [Mate]: Abstandshalter 14mm leicht:1 ↔ Gewindestange M3x85mm:2
- Passend:381 [Mate]: Abstandshalter 14mm leicht:4 ↔ Gewindestange M3x85mm:2
- Passend:382 [Mate]: Abstandshalter 14mm leicht:1 ↔ Halterung Lichtschranke rechts:1
- Passend:383 [Mate]: Abstandshalter 14mm leicht:4 ↔ Halterung Lichtschranke rechts:2
- Passend:384 [Mate]: Abstandshalter 14mm leicht:3 ↔ Halterung Lichtschranke links:1
- Passend:385 [Mate]: Abstandshalter 14mm leicht:2 ↔ Halterung Lichtschranke links:2
- Passend:386 [Mate]: Abstandshalter 14mm leicht:3 ↔ Halterung Lichtschranke links:2
- Passend:387 [Mate]: Abstandshalter 14mm leicht:2 ↔ Halterung Lichtschranke links:3
- Passend:388 [Mate]: Akkuhalterung:2 ↔ Pixy 2 Halterung:1
- Passend:389 [Mate]: Sicherungsmutter M3:24 ↔ Gewindestange M3x85mm:1
- Passend:390 [Mate]: Sicherungsmutter M3:25 ↔ Gewindestange M3x85mm:2
- Passend:391 [Mate]: Sicherungsmutter M3:24 ↔ Pixy 2 Halterung:1
- Passend:392 [Mate]: Sicherungsmutter M3:25 ↔ Pixy 2 Halterung:1
- Passend:393 [Mate]: Schraube M3x16 LK:9 ↔ Motorhalterung leicht VR:1
- Passend:394 [Mate]: Schraube M3x16 LK:9 ↔ Hauptplatine:1
- Passend:395 [Mate]: Scheibe M3 Polyamid:27 ↔ Hauptplatine:1
- Passend:396 [Mate]: Scheibe M3 Polyamid:27 ↔ Hauptplatine:1
- Passend:397 [Mate]: Schraube M3x16 LK:9 ↔ Scheibe M3 Polyamid:27
- Passend:398 [Mate]: Bodenplatine:1 ↔ Scheibe M3 Polyamid:23
- Passend:399 [Mate]: Schraube M3x16 LK:8 ↔ Scheibe M3 Polyamid:23
- Passend:400 [Mate]: Schraube M3x16 LK:8 ↔ Scheibe M3 Polyamid:23
- Passend:401 [Mate]: Schraube M3x12 LK:1 ↔ Pixy 2 Halterung:1
- Passend:404 [Mate]: Sicherungsmutter M3:27 ↔ Schraube M3x12 LK:1
- Passend:405 [Mate]: Sicherungsmutter M3:26 ↔ Schraube M3x12 LK:2
- Passend:406 [Mate]: Sicherungsmutter M3:28 ↔ Schraube M3x12 LK:3
- Passend:407 [Mate]: Sicherungsmutter M3:27 ↔ Pixy 2 Halterung:1
- Passend:408 [Mate]: Sicherungsmutter M3:26 ↔ Pixy 2 Halterung:1
- Passend:409 [Mate]: Sicherungsmutter M3:28 ↔ Pixy 2 Halterung:1
